# Autodesk Inventor assembly: E001_BancDeTest
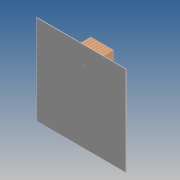
[picture p0: Inventor's stored thumbnail of the model, 180x180]
Saved by Autodesk Inventor 2020 (Build 240168000, 168)
## iProperties
Created: 2021-09-24
Part Number: E001_BancDeTest
Document SubType Name: Assembly
Designer: gabri
Author: gabri
## Documents named in this file (4)
- D:\PGA\E001_BancDeTest.iam
- D:\PGA\P002_plancher.ipt
- D:\PGA\P001_CageDeTest.ipt
- D:\PGA\P003_tripod.ipt
## Components (3 placed, 3 different names)
1. P002_plancher:1 — Placage:1, Placage:2, Placage:3, Placage:4, Placage:5
2. P001_CageDeTest:1 — Placage:4
3. P003_tripod:1 — Placage:5
## Relationships (5: Mate 5)
- Placage:1 [Mate]: P002_plancher:1
- Placage:2 [Mate]: P002_plancher:1
- Placage:3 [Mate]: P002_plancher:1
- Placage:4 [Mate]: P002_plancher:1 ↔ P001_CageDeTest:1
- Placage:5 [Mate] (900 mm): P002_plancher:1 ↔ P003_tripod:1
